# Autodesk Inventor assembly: Cart
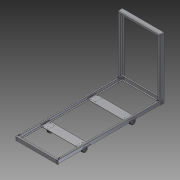
[picture p0: Inventor's stored thumbnail of the model, 180x180]
Saved by Autodesk Inventor 2012 (Build 160160000, 160)
## iProperties
Created: 2011-10-13
Part Number: Cart
Document SubType Name: Assembly
Designer: Tushar
Author: Tushar
## Documents named in this file (9)
- C:\Users\Tushar\Dropbox\CAD Inventor\Preseason Projects\Cart Competition Cart\Sah\Cart.iam
- C:\Users\Tushar\Dropbox\CAD Inventor\Preseason Projects\Cart Competition Cart\Sah\Base Side Bar.ipt
- C:\Users\Tushar\Dropbox\CAD Inventor\Preseason Projects\Cart Competition Cart\Sah\Base Back Bar.ipt
- C:\Users\Tushar\Dropbox\CAD Inventor\Preseason Projects\Cart Competition Cart\Sah\Base Top.ipt
- C:\Users\Tushar\Dropbox\CAD Inventor\Preseason Projects\Cart Competition Cart\Sah\Base Crossbar.ipt
- C:\Users\Tushar\Dropbox\CAD Inventor\Preseason Projects\Cart Competition Cart\Sah\Handle Bar.ipt
- C:\Users\Tushar\Dropbox\CAD Inventor\Preseason Projects\Cart Competition Cart\Sah\IFI 114 - .125  x .27.ipt
- C:\Users\Tushar\Dropbox\CAD Inventor\Preseason Projects\Cart Competition Cart\Sah\IFI 114 - .125  x .36.ipt
- C:\Users\Tushar\Dropbox\CAD Inventor\Preseason Projects\Cart Competition Cart\Sah\Caster\goalcaster.iam
## Components (100 placed, 8 different names)
1. Base Side Bar:1 — Mate:1, Flush:1, Mate:2, Mate:9, Flush:5, Mate:11, Mate:15, Mate:17, Mate:33, Mate:34, Mate:40, Mate:42, Mate:43, Flush:19, Mate:50
2. Base Side Bar:2 — Mate:3, Mate:4, Flush:2, Mate:5, Mate:6, Mate:7, Mate:8, Flush:7, Flush:11, Mate:39, Mate:41
3. Base Back Bar:1 — Mate:1, Flush:1, Mate:2, Mate:3, Mate:4, Flush:2, Mate:10, Mate:12, Mate:44
4. Base Top:1 — Mate:9, Flush:5, Mate:13, Mate:28, Mate:29, Mate:30, Mate:31, Mate:32, Mate:44, Mate:45, Mate:46, Mate:47, Mate:48, Mate:49
5. Base Crossbar:1 — Mate:6, Mate:7, Flush:11, Mate:35, Mate:36, Flush:15, Flush:16
6. Base Crossbar:2 — Mate:5, Mate:8, Flush:7, Mate:37, Mate:38, Flush:20, Flush:21
7. Handle Bar:1 — Mate:10, Mate:11, Mate:12, Mate:13, Mate:18, Mate:19, Mate:20, Mate:21, Mate:22, Mate:23, Mate:24, Mate:25, Mate:26, Mate:27
8. Base Back Bar:2 — Mate:43, Flush:19, Mate:50, Mate:51, Mate:52
9. IFI 114 - .1875  x .27:64 — Mate:28, Flush:8, Flush:9, Flush:10, Mate:32
10. IFI 114 - .1875  x .27:65 — Mate:29, Flush:8
11. IFI 114 - .1875  x .27:66 — Mate:30, Flush:9
12. IFI 114 - .1875  x .27:67 — Mate:31, Flush:10
13. IFI 114 - .1875  x .27:107
14. IFI 114 - .1875  x .27:108
15. IFI 114 - .1875  x .27:109
16. IFI 114 - .1875  x .27:70
17. IFI 114 - .1875  x .27:71
18. IFI 114 - .1875  x .27:72
19. IFI 114 - .1875  x .27:73
20. IFI 114 - .1875  x .27:74
21. IFI 114 - .1875  x .27:75
22. IFI 114 - .1875  x .27:76
23. IFI 114 - .1875  x .27:77
24. IFI 114 - .1875  x .27:78
25. IFI 114 - .1875  x .27:79
26. IFI 114 - .1875  x .27:80
27. IFI 114 - .1875  x .27:81
28. IFI 114 - .1875  x .27:82
29. IFI 114 - .1875  x .27:83
30. IFI 114 - .1875  x .27:84
31. IFI 114 - .1875  x .27:85
32. IFI 114 - .1875  x .27:86
33. IFI 114 - .1875  x .27:87
34. IFI 114 - .1875  x .27:88
35. IFI 114 - .1875  x .27:89
36. IFI 114 - .1875  x .27:90
37. IFI 114 - .1875  x .27:91
38. IFI 114 - .1875  x .27:92
39. IFI 114 - .125  x .36:8
40. IFI 114 - .125  x .36:9
41. IFI 114 - .125  x .36:10
42. IFI 114 - .1875  x .27:93
43. IFI 114 - .1875  x .27:94
44. IFI 114 - .1875  x .27:95
45. IFI 114 - .125  x .36:11
46. IFI 114 - .125  x .36:12
47. IFI 114 - .125  x .36:13
48. IFI 114 - .125  x .36:14
49. IFI 114 - .1875  x .27:96
50. IFI 114 - .1875  x .27:97
51. IFI 114 - .1875  x .27:98 — Flush:12, Flush:13, Flush:14, Mate:45, Mate:49
52. IFI 114 - .1875  x .27:99 — Flush:12, Mate:47
53. IFI 114 - .1875  x .27:100 — Flush:13, Mate:46
54. IFI 114 - .1875  x .27:101 — Flush:14, Mate:48
55. IFI 114 - .1875  x .27:102
56. IFI 114 - .1875  x .27:103
57. goalcaster:1 [sub-assembly] — Mate:35, Flush:16, Mate:39
58. goalcaster:2 [sub-assembly] — Mate:36, Flush:15, Mate:40
59. goalcaster:3 [sub-assembly] — Mate:37, Mate:41, Flush:21
60. goalcaster:4 [sub-assembly] — Mate:38, Mate:42, Flush:20
61. IFI 114 - .1875  x .27:1 — Mate:15, Mate:33
62. IFI 114 - .1875  x .27:2
63. IFI 114 - .1875  x .27:3
64. IFI 114 - .1875  x .27:4
65. IFI 114 - .1875  x .27:5
66. IFI 114 - .1875  x .27:6
67. IFI 114 - .1875  x .27:7
68. IFI 114 - .1875  x .27:68
69. IFI 114 - .1875  x .27:69
70. IFI 114 - .1875  x .27:15 — Mate:17, Mate:34
71. IFI 114 - .1875  x .27:16
72. IFI 114 - .1875  x .27:17
73. IFI 114 - .1875  x .27:18
74. IFI 114 - .1875  x .27:19
75. IFI 114 - .1875  x .27:20
76. IFI 114 - .1875  x .27:21
77. IFI 114 - .1875  x .27:22 — Mate:18, Mate:19
78. IFI 114 - .1875  x .27:23
79. IFI 114 - .1875  x .27:24
80. IFI 114 - .1875  x .27:25
81. IFI 114 - .1875  x .27:26
82. IFI 114 - .1875  x .27:27
83. IFI 114 - .1875  x .27:28
84. IFI 114 - .1875  x .27:29
85. IFI 114 - .1875  x .27:30
86. IFI 114 - .125  x .36:1 — Mate:20, Mate:21
87. IFI 114 - .125  x .36:2
88. IFI 114 - .125  x .36:3
89. IFI 114 - .1875  x .27:31 — Mate:22, Mate:23
90. IFI 114 - .1875  x .27:32
91. IFI 114 - .1875  x .27:33
92. IFI 114 - .125  x .36:4 — Mate:24, Mate:25
93. IFI 114 - .125  x .36:5
94. IFI 114 - .125  x .36:6
95. IFI 114 - .125  x .36:7
96. IFI 114 - .1875  x .27:34 — Mate:26, Mate:27
97. IFI 114 - .1875  x .27:35
98. IFI 114 - .1875  x .27:104 — Mate:51, Mate:52
99. IFI 114 - .1875  x .27:105
100. IFI 114 - .1875  x .27:106
## Component patterns: (9 elements, first: IFI 114 - .1875  x .27:1), (7 elements, first: IFI 114 - .1875  x .27:15), (9 elements, first: IFI 114 - .1875  x .27:22), (3 elements, first: IFI 114 - .125  x .36:1), (3 elements, first: IFI 114 - .1875  x .27:31), (4 elements, first: IFI 114 - .125  x .36:4), (2 elements, first: IFI 114 - .1875  x .27:34), (3 elements, first: IFI 114 - .1875  x .27:104)
## Relationships (66: Mate 50, Flush 16)
- Mate:1: Base Side Bar:1 ↔ Base Back Bar:1
- Flush:1: Base Side Bar:1 ↔ Base Back Bar:1
- Mate:2: Base Side Bar:1 ↔ Base Back Bar:1
- Mate:3: Base Side Bar:2 ↔ Base Back Bar:1
- Mate:4: Base Side Bar:2 ↔ Base Back Bar:1
- Flush:2: Base Side Bar:2 ↔ Base Back Bar:1
- Mate:5: Base Side Bar:2 ↔ Base Crossbar:2
- Mate:6: Base Side Bar:2 ↔ Base Crossbar:1
- Mate:7: Base Side Bar:2 ↔ Base Crossbar:1
- Mate:8: Base Side Bar:2 ↔ Base Crossbar:2
- Mate:9: Base Side Bar:1 ↔ Base Top:1
- Flush:5: Base Side Bar:1 ↔ Base Top:1
- Mate:10: Base Back Bar:1 ↔ Handle Bar:1
- Mate:11: Base Side Bar:1 ↔ Handle Bar:1
- Mate:12: Base Back Bar:1 ↔ Handle Bar:1
- Mate:13: Base Top:1 ↔ Handle Bar:1
- Flush:7 (-381 mm): Base Side Bar:2 ↔ Base Crossbar:2
- Mate:15: Base Side Bar:1 ↔ IFI 114 - .1875  x .27:1
- Mate:17: Base Side Bar:1 ↔ IFI 114 - .1875  x .27:15
- Mate:18: Handle Bar:1 ↔ IFI 114 - .1875  x .27:22
- Mate:19: Handle Bar:1 ↔ IFI 114 - .1875  x .27:22
- Mate:20: Handle Bar:1 ↔ IFI 114 - .125  x .36:1
- Mate:21: Handle Bar:1 ↔ IFI 114 - .125  x .36:1
- Mate:22: Handle Bar:1 ↔ IFI 114 - .1875  x .27:31
- Mate:23: Handle Bar:1 ↔ IFI 114 - .1875  x .27:31
- Mate:24: Handle Bar:1 ↔ IFI 114 - .125  x .36:4
- Mate:25: Handle Bar:1 ↔ IFI 114 - .125  x .36:4
- Mate:26: Handle Bar:1 ↔ IFI 114 - .1875  x .27:34
- Mate:27: Handle Bar:1 ↔ IFI 114 - .1875  x .27:34
- Mate:28: Base Top:1 ↔ IFI 114 - .1875  x .27:64
- Mate:29: Base Top:1 ↔ IFI 114 - .1875  x .27:65
- Mate:30: Base Top:1 ↔ IFI 114 - .1875  x .27:66
- Mate:31: Base Top:1 ↔ IFI 114 - .1875  x .27:67
- Flush:8: IFI 114 - .1875  x .27:64 ↔ IFI 114 - .1875  x .27:65
- Flush:9: IFI 114 - .1875  x .27:64 ↔ IFI 114 - .1875  x .27:66
- Flush:10: IFI 114 - .1875  x .27:64 ↔ IFI 114 - .1875  x .27:67
- Mate:32: Base Top:1 ↔ IFI 114 - .1875  x .27:64
- Flush:11 (-355.6 mm): Base Side Bar:2 ↔ Base Crossbar:1
- Mate:33: Base Side Bar:1 ↔ IFI 114 - .1875  x .27:1
- Mate:34: Base Side Bar:1 ↔ IFI 114 - .1875  x .27:15
- Flush:12: IFI 114 - .1875  x .27:98 ↔ IFI 114 - .1875  x .27:99
- Flush:13: IFI 114 - .1875  x .27:98 ↔ IFI 114 - .1875  x .27:100
- Flush:14: IFI 114 - .1875  x .27:98 ↔ IFI 114 - .1875  x .27:101
- Mate:35: Base Crossbar:1 ↔ goalcaster:1
- Mate:36: Base Crossbar:1 ↔ goalcaster:2
- Mate:37: Base Crossbar:2 ↔ goalcaster:3
- Mate:38: Base Crossbar:2 ↔ goalcaster:4
- Flush:15: Base Crossbar:1 ↔ goalcaster:2
- Flush:16: Base Crossbar:1 ↔ goalcaster:1
- Mate:39: Base Side Bar:2 ↔ goalcaster:1
- Mate:40: Base Side Bar:1 ↔ goalcaster:2
- Mate:41: Base Side Bar:2 ↔ goalcaster:3
- Mate:42: Base Side Bar:1 ↔ goalcaster:4
- Mate:43: Base Side Bar:1 ↔ Base Back Bar:2
- Mate:44: Base Back Bar:1 ↔ Base Top:1
- Mate:45: Base Top:1 ↔ IFI 114 - .1875  x .27:98
- Mate:46: Base Top:1 ↔ IFI 114 - .1875  x .27:100
- Mate:47: Base Top:1 ↔ IFI 114 - .1875  x .27:99
- Mate:48: Base Top:1 ↔ IFI 114 - .1875  x .27:101
- Mate:49: Base Top:1 ↔ IFI 114 - .1875  x .27:98
- Flush:19: Base Side Bar:1 ↔ Base Back Bar:2
- Mate:50: Base Side Bar:1 ↔ Base Back Bar:2
- Mate:51: Base Back Bar:2 ↔ IFI 114 - .1875  x .27:104
- Mate:52: Base Back Bar:2 ↔ IFI 114 - .1875  x .27:104
- Flush:20: Base Crossbar:2 ↔ goalcaster:4
- Flush:21: Base Crossbar:2 ↔ goalcaster:3
